# Autodesk Inventor assembly: ASY ANP 1426 FDS way 6
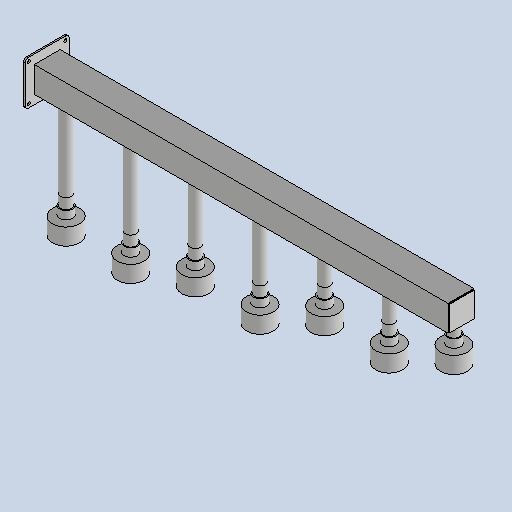
[picture p0: Inventor's stored thumbnail of the model, 512x512]
Saved by Autodesk Inventor 2025 (Build 290162010, 162A)
## iProperties
Created: 2025-07-02
Part Number: ASY ANP 1426 FDS way 6
Document SubType Name: Assembly
Designer: admin
Author: user
## Documents named in this file (9)
- C:\Users\pokla\Documents\Inventor\ANP--Antipayuta\FDS 1400\ASY ANP 1426 FDS way 6.iam
- C:\Users\pokla\Documents\Inventor\ANP--Antipayuta\FDS 1400\ANP 1436 FDS WAY tube6.ipt
- C:\Users\pokla\Documents\Inventor\ANP--Antipayuta\FDS 1400\ANP 1425 FDS Way FLANGE.ipt
- C:\Users\pokla\Documents\Inventor\ANP--Antipayuta\FDS 1400\ANP 1426 FDS way cup.ipt
- C:\Users\pokla\Documents\Inventor\ANP--Antipayuta\FDS 1400\ANP dummy filter element.ipt
- C:\Users\pokla\Documents\Inventor\ANP--Antipayuta\FDS 1400\ANP dummy pipe nippel.ipt
- C:\Users\pokla\Documents\Inventor\ANP--Antipayuta\FDS 1400\ANP 1448 FDS thread  tube8.ipt
- C:\Users\pokla\Documents\Inventor\ANP--Antipayuta\FDS 1400\ANP 1449 FDS thread  tube9.ipt
- C:\Users\pokla\Documents\Inventor\ANP--Antipayuta\FDS 1400\ANP 1451 FDS thread  tube10.ipt
## Components (23 placed, 8 different names)
1. TKS 3536 FDS WAY tube6:1 — Rigid:34, Rigid:35, Rigid:36, Rigid:53, Rigid:54, Rigid:55, Rigid:26, Rigid:27, Rigid:28
2. TKS 3525 FDS Way FLANGE:1 — Rigid:34
3. TKS 3526 FDS way cup:1 — Rigid:35
4. TKS dummy filter element:1 — Rigid:1
5. TKS dummy pipe nippel:1 — Rigid:1, Rigid:44
6. TKS dummy filter element:2 — Rigid:6
7. TKS dummy pipe nippel:2 — Rigid:6, Rigid:46
8. TKS dummy filter element:3 — Rigid:14
9. TKS dummy pipe nippel:3 — Rigid:14, Rigid:45
10. TKS dummy filter element:4 — Rigid:33
11. TKS dummy pipe nippel:4 — Rigid:36, Rigid:33
12. TKS 3548 FDS thread  tube8:1 — Rigid:53, Rigid:46
13. TKS 3549 FDS thread  tube9:1 — Rigid:54, Rigid:45
14. TKS 3551 FDS thread  tube10:1 — Rigid:55, Rigid:44
15. TKS dummy filter element:5
16. TKS dummy pipe nippel:5
17. TKS dummy filter element:6
18. TKS dummy pipe nippel:6
19. TKS 3548 FDS thread  tube8:2 — Rigid:28
20. TKS 3549 FDS thread  tube9:2 — Rigid:27
21. TKS dummy filter element:7
22. TKS dummy pipe nippel:7
23. TKS 3551 FDS thread  tube10:2 — Rigid:26
## Relationships (22: WeldJoint 22)
- Rigid:34 [WeldJoint] (2 mm): TKS 3536 FDS WAY tube6:1 ↔ TKS 3525 FDS Way FLANGE:1
- Rigid:35 [WeldJoint]: TKS 3536 FDS WAY tube6:1 ↔ TKS 3526 FDS way cup:1
- Rigid:1 [WeldJoint]: TKS dummy filter element:1 ↔ TKS dummy pipe nippel:1
- Rigid:6 [WeldJoint]: TKS dummy filter element:2 ↔ TKS dummy pipe nippel:2
- Rigid:14 [WeldJoint]: TKS dummy filter element:3 ↔ TKS dummy pipe nippel:3
- Rigid:36 [WeldJoint]: TKS 3536 FDS WAY tube6:1 ↔ TKS dummy pipe nippel:4
- Rigid:33 [WeldJoint]: TKS dummy filter element:4 ↔ TKS dummy pipe nippel:4
- Rigid:53 [WeldJoint]: TKS 3536 FDS WAY tube6:1 ↔ TKS 3548 FDS thread  tube8:1
- Rigid:46 [WeldJoint]: TKS dummy pipe nippel:2 ↔ TKS 3548 FDS thread  tube8:1
- Rigid:54 [WeldJoint]: TKS 3536 FDS WAY tube6:1 ↔ TKS 3549 FDS thread  tube9:1
- Rigid:45 [WeldJoint]: TKS dummy pipe nippel:3 ↔ TKS 3549 FDS thread  tube9:1
- Rigid:55 [WeldJoint]: TKS 3536 FDS WAY tube6:1 ↔ TKS 3551 FDS thread  tube10:1
- Rigid:44 [WeldJoint]: TKS dummy pipe nippel:1 ↔ TKS 3551 FDS thread  tube10:1
- [WeldJoint]: TKS dummy filter element:5 ↔ TKS dummy pipe nippel:5
- [WeldJoint]: TKS dummy filter element:6 ↔ TKS dummy pipe nippel:6
- [WeldJoint]: TKS dummy pipe nippel:5 ↔ TKS 3548 FDS thread  tube8:2
- [WeldJoint]: TKS dummy pipe nippel:6 ↔ TKS 3549 FDS thread  tube9:2
- [WeldJoint]: TKS dummy filter element:7 ↔ TKS dummy pipe nippel:7
- [WeldJoint]: TKS dummy pipe nippel:7 ↔ TKS 3551 FDS thread  tube10:2
- Rigid:26 [WeldJoint]: TKS 3536 FDS WAY tube6:1 ↔ TKS 3551 FDS thread  tube10:2
- Rigid:27 [WeldJoint]: TKS 3536 FDS WAY tube6:1 ↔ TKS 3549 FDS thread  tube9:2
- Rigid:28 [WeldJoint]: TKS 3536 FDS WAY tube6:1 ↔ TKS 3548 FDS thread  tube8:2
## Named parameters: d25_d14 = 0 mm, d26_d16 = 0 mm, d27_d3 = 0 mm, d28_d5 = 0 mm, d29_d18 = 0 mm, d30_d2 = 0 mm
